# Autodesk Inventor assembly: 3DCP-NOZZLEv2
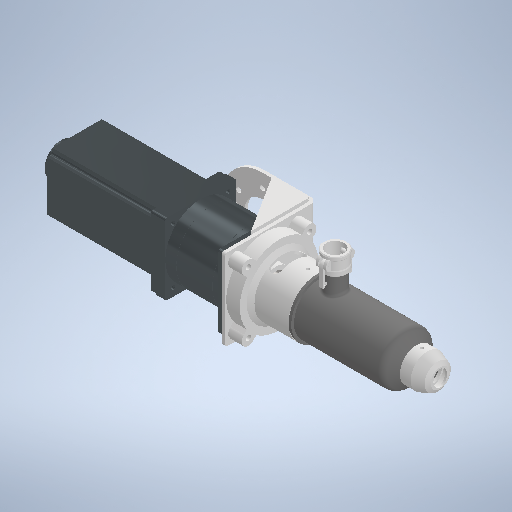
[picture p0: Inventor's stored thumbnail of the model, 512x512]
Saved by Autodesk Inventor 2025.4 (Build 294407000, 407)
## iProperties
Created: 2025-09-28
Part Number: 3DCP-NOZZLEv2
Document SubType Name: Assembly
Designer: lstk1ng
Description: 3DCP NOZZLE
Mass: 20044.7 g
Surface Area: 7725.76 cm^2
Volume: 5908.78 cm^3
Density: 3.39236 g/cm^3
Author: lstk1ng
## Documents named in this file (11)
- C:\Users\K1NG\Documents\PM2 archives\DISEÑO MECANICO-v2\DISEÑO MECANICO\3DCP-NOZZLEv2.iam
- C:\Users\K1NG\Documents\PM2 archives\DISEÑO MECANICO-v2\DISEÑO MECANICO\COMPONENTS\MEZCLADOR-TRUPPER-80MM.ipt
- C:\Users\K1NG\Documents\PM2 archives\DISEÑO MECANICO-v2\DISEÑO MECANICO\COMPONENTS\PX130-GEARBOX.ipt
- C:\Users\K1NG\Documents\PM2 archives\DISEÑO MECANICO-v2\DISEÑO MECANICO\COMPONENTS\SERVOMOTOR-2.3KWv1.ipt
- C:\Users\K1NG\Documents\PM2 archives\DISEÑO MECANICO-v2\DISEÑO MECANICO\M20 x 80.ipt
- C:\Users\K1NG\Documents\PM2 archives\DISEÑO MECANICO-v2\DISEÑO MECANICO\COMPONENTS\JAW-COUPLING-ID22MM.iam
- C:\Users\K1NG\Documents\PM2 archives\DISEÑO MECANICO-v2\DISEÑO MECANICO\NOZZLE-FLANGE.ipt
- C:\Users\K1NG\Documents\PM2 archives\DISEÑO MECANICO-v2\DISEÑO MECANICO\NOZZLES\NOZZLE-ELIPTICO.ipt
- C:\Users\K1NG\Documents\PM2 archives\DISEÑO MECANICO-v2\DISEÑO MECANICO\LOWER-NOZZLEv3.ipt
- C:\Users\K1NG\Documents\PM2 archives\DISEÑO MECANICO-v2\DISEÑO MECANICO\UPPER-NOZZLEvF2.0.ipt
- C:\Users\K1NG\Documents\PM2 archives\DISEÑO MECANICO-v2\DISEÑO MECANICO\COMPONENTS\CAMLOCK TIPO B 3'4IN.ipt
## Components (10 placed, 10 different names)
1. MEZCLADOR-TRUPPER-80MM:1 — Mate:1, Mate:2, Mate:3
2. PX130-GEARBOX:1 — Mate:6, Mate:7, Mate:8, Mate:10, Mate:11, Mate:12, Mate:43, Mate:44, Mate:49
3. SERVOMOTOR-2.3KWv1:1 — Mate:6, Mate:7, Mate:10
4. AS 1110 - Metric M20 x 80:1 — Mate:1, Mate:2, Mate:3, Mate:4, Mate:5
5. JAW-COUPLING-ID22MM:1 [sub-assembly] — Mate:4, Mate:5, Mate:43, Mate:50
6. NOZZLE-FLANGE:1 — Mate:8, Mate:11, Mate:12, Mate:27, Mate:28, Mate:29, Mate:30, Mate:31, Mate:33
7. NOZZLE-ELIPTICO:1 — Mate:54, Mate:55, Mate:59
8. LOWER-NOZZLEv3:1 — Mate:44, Mate:51, Mate:55, Mate:57, Mate:58, Mate:59
9. UPPER-NOZZLEvF2.0:1 — Mate:49, Mate:50, Mate:51, Mate:54, Mate:58
10. CAMLOCK TIPO B 3'4IN:1 — Mate:57
## Relationships (27: Mate 27)
- Mate:1: MEZCLADOR-TRUPPER-80MM:1 ↔ AS 1110 - Metric M20 x 80:1
- Mate:2: MEZCLADOR-TRUPPER-80MM:1 ↔ AS 1110 - Metric M20 x 80:1
- Mate:3: MEZCLADOR-TRUPPER-80MM:1 ↔ AS 1110 - Metric M20 x 80:1
- Mate:4: AS 1110 - Metric M20 x 80:1 ↔ JAW-COUPLING-ID22MM:1
- Mate:5: AS 1110 - Metric M20 x 80:1 ↔ JAW-COUPLING-ID22MM:1
- Mate:6: PX130-GEARBOX:1 ↔ SERVOMOTOR-2.3KWv1:1
- Mate:7: PX130-GEARBOX:1 ↔ SERVOMOTOR-2.3KWv1:1
- Mate:8: PX130-GEARBOX:1 ↔ NOZZLE-FLANGE:1
- Mate:10: PX130-GEARBOX:1 ↔ SERVOMOTOR-2.3KWv1:1
- Mate:11: PX130-GEARBOX:1 ↔ NOZZLE-FLANGE:1
- Mate:12: PX130-GEARBOX:1 ↔ NOZZLE-FLANGE:1
- Mate:27: NOZZLE-FLANGE:1
- Mate:28: NOZZLE-FLANGE:1
- Mate:29: NOZZLE-FLANGE:1
- Mate:30: NOZZLE-FLANGE:1
- Mate:31: NOZZLE-FLANGE:1
- Mate:33: NOZZLE-FLANGE:1
- Mate:43: PX130-GEARBOX:1 ↔ JAW-COUPLING-ID22MM:1
- Mate:44: PX130-GEARBOX:1 ↔ LOWER-NOZZLEv3:1
- Mate:49: PX130-GEARBOX:1 ↔ UPPER-NOZZLEvF2.0:1
- Mate:50: JAW-COUPLING-ID22MM:1 ↔ UPPER-NOZZLEvF2.0:1
- Mate:51: LOWER-NOZZLEv3:1 ↔ UPPER-NOZZLEvF2.0:1
- Mate:54: NOZZLE-ELIPTICO:1 ↔ UPPER-NOZZLEvF2.0:1
- Mate:55: NOZZLE-ELIPTICO:1 ↔ LOWER-NOZZLEv3:1
- Mate:57: LOWER-NOZZLEv3:1 ↔ CAMLOCK TIPO B 3'4IN:1
- Mate:58: LOWER-NOZZLEv3:1 ↔ UPPER-NOZZLEvF2.0:1
- Mate:59: NOZZLE-ELIPTICO:1 ↔ LOWER-NOZZLEv3:1
